# Autodesk Inventor assembly: wheel_assm
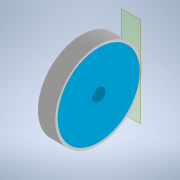
[picture p0: Inventor's stored thumbnail of the model, 180x180]
Saved by Autodesk Inventor 2020 (Build 240168000, 168)
## iProperties
Created: 2020-06-07
Part Number: wheel_assm
Document SubType Name: Assembly
Designer: Abhinav Roy
Author: Abhinav Roy
## Documents named in this file (3)
- D:\Mopping_Robot\cad\V1.0\wheel_assm.iam
- D:\Mopping_Robot\cad\V1.0\wheel.ipt
- D:\Mopping_Robot\cad\V1.0\silicon_sheath.ipt
## Components (2 placed, 2 different names)
1. wheel:1 — Flush:1, Mate:1
2. silicon_sheath:1 — Flush:1, Mate:1
## Relationships (2: Flush 1, Mate 1)
- Flush:1: wheel:1 ↔ silicon_sheath:1
- Mate:1: wheel:1 ↔ silicon_sheath:1
